# Autodesk Inventor assembly: CaseAssembly
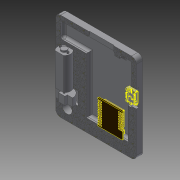
[picture p0: Inventor's stored thumbnail of the model, 180x180]
Saved by Autodesk Inventor 2015 SP2 (Build 190223200, 223)
## iProperties
Created: 2016-07-20
Part Number: CaseAssembly
Document SubType Name: Assembly
Designer: Iain
Author: Iain
## Documents named in this file (4)
- D:\Sit-To-Stand\BLEVibrator\Hardware\Case\CaseAssembly.iam
- D:\Sit-To-Stand\BLEVibrator\Hardware\Case\308-106.ipt
- D:\Sit-To-Stand\BLEVibrator\Hardware\Case\CaseBase.ipt
- D:\Sit-To-Stand\BLEVibrator\Hardware\Case\PCBAssembly.iam
## Components (3 placed, 3 different names)
1. 308-106:1 — Insert:1
2. CaseBase:1 — Mate:1, Flush:1, Flush:2, Insert:1
3. PCBAssembly:1 [sub-assembly] — Mate:1, Flush:1, Flush:2
## Relationships (4: Flush 2, Mate 1, Insert 1)
- Mate:1: CaseBase:1 ↔ PCBAssembly:1
- Flush:1 (0.5 mm): CaseBase:1 ↔ PCBAssembly:1
- Flush:2 (0.7 mm): CaseBase:1 ↔ PCBAssembly:1
- Insert:1 (1.1 mm): 308-106:1 ↔ CaseBase:1
